# Autodesk Inventor assembly: 4C
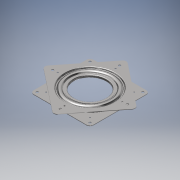
[picture p0: Inventor's stored thumbnail of the model, 180x180]
Saved by Autodesk Inventor 2017.1 (Build 211199000, 199)
## iProperties
Company: Autodesk Inc.
Category: Loose
Created: 2016-12-24
Part Number: 4C
Document SubType Name: Assembly
Designer: Autodesk Inc.
Catalog Web Link: http://www.triangleoshkosh.com/products/en/4-ungreased-lazy-susan-bearing
Vendor: Triangle Mfg.
Author: Autodesk Inc.
Keywords: Gray Tote
## Documents named in this file (4)
- D:\FIRST\FIRST KOP 2017\FIRST 2017 Gray Tote\LazySusan_4C.iam
- D:\FIRST\FIRST KOP 2017\FIRST 2017 Gray Tote\Parts\MSTR 4 Inch Locking Race_7719a.ipt
- D:\FIRST\FIRST KOP 2017\FIRST 2017 Gray Tote\Parts\MSTR 4 Inch Plain Race_2823.ipt
- D:\FIRST\FIRST KOP 2017\FIRST 2017 Gray Tote\Parts\MSTR Suzie Ball_Balls4.ipt
## Components (38 placed, 38 different names)
1. MSTR 4 Inch Locking Race_7719a_1 — Mate:1, Mate:2
2. MSTR 4 Inch Plain Race_2823_2 — Mate:1, Mate:2
3. MSTR Suzie Ball_Balls4_3
4. MSTR Suzie Ball_Balls4_4
5. MSTR Suzie Ball_Balls4_5
6. MSTR Suzie Ball_Balls4_6
7. MSTR Suzie Ball_Balls4_7
8. MSTR Suzie Ball_Balls4_8
9. MSTR Suzie Ball_Balls4_9
10. MSTR Suzie Ball_Balls4_10
11. MSTR Suzie Ball_Balls4_11
12. MSTR Suzie Ball_Balls4_12
13. MSTR Suzie Ball_Balls4_13
14. MSTR Suzie Ball_Balls4_14
15. MSTR Suzie Ball_Balls4_15
16. MSTR Suzie Ball_Balls4_16
17. MSTR Suzie Ball_Balls4_17
18. MSTR Suzie Ball_Balls4_18
19. MSTR Suzie Ball_Balls4_19
20. MSTR Suzie Ball_Balls4_20
21. MSTR Suzie Ball_Balls4_21
22. MSTR Suzie Ball_Balls4_22
23. MSTR Suzie Ball_Balls4_23
24. MSTR Suzie Ball_Balls4_24
25. MSTR Suzie Ball_Balls4_25
26. MSTR Suzie Ball_Balls4_26
27. MSTR Suzie Ball_Balls4_27
28. MSTR Suzie Ball_Balls4_28
29. MSTR Suzie Ball_Balls4_29
30. MSTR Suzie Ball_Balls4_30
31. MSTR Suzie Ball_Balls4_31
32. MSTR Suzie Ball_Balls4_32
33. MSTR Suzie Ball_Balls4_33
34. MSTR Suzie Ball_Balls4_34
35. MSTR Suzie Ball_Balls4_35
36. MSTR Suzie Ball_Balls4_36
37. MSTR Suzie Ball_Balls4_37
38. MSTR Suzie Ball_Balls4_38
## Relationships (2: Mate 2)
- Mate:1: MSTR 4 Inch Locking Race_7719a_1 ↔ MSTR 4 Inch Plain Race_2823_2
- Mate:2 (6.6548 mm): MSTR 4 Inch Locking Race_7719a_1 ↔ MSTR 4 Inch Plain Race_2823_2
